# Autodesk Inventor assembly: Gear central part
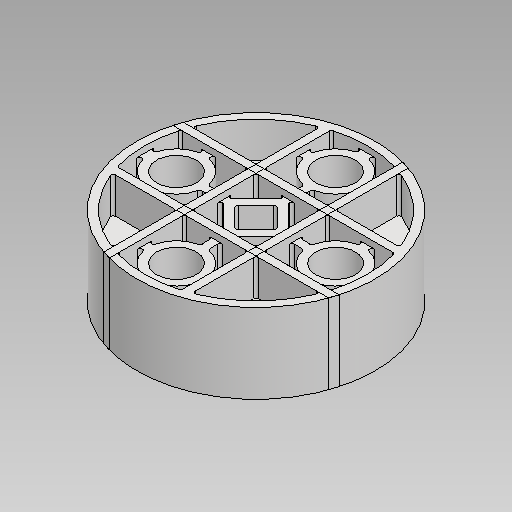
[picture p0: Inventor's stored thumbnail of the model, 512x512]
Saved by Autodesk Inventor 2020 (Build 240168000, 168)
## iProperties
Created: 2019-05-06
Part Number: Gear central part
Document SubType Name: Assembly
Designer: Varga Daniel
Author: Varga Daniel
## Documents named in this file (3)
- C:\!_Dani\!_cloud\OneDrive\!_munka\Revolution\StructuralParts\Gears\Gear central part.iam
- C:\!_Dani\!_cloud\OneDrive\!_munka\Revolution\StructuralParts\Gears\Gear side part.ipt
- C:\!_Dani\!_cloud\OneDrive\!_munka\Revolution\StructuralParts\Beams\Axle Beams\Axle beam base.ipt
## Components (5 placed, 2 different names)
1. Gear side part:1 — Flush:4, Flush:8, Flush:11
2. Gear side part:2 — Flush:2, Flush:6, Flush:9
3. Gear side part:3 — Flush:1, Flush:5, Flush:12
4. Gear side part:4 — Flush:3, Flush:7, Flush:10
5. Axle beam base:1 — Flush:1, Flush:2, Flush:3, Flush:4, Flush:5, Flush:6, Flush:7, Flush:8, Flush:9, Flush:10, Flush:11, Flush:12, Mate:1, Mate:2, Flush:13
## Relationships (15: Flush 13, Mate 2)
- Flush:1: Gear side part:3 ↔ Axle beam base:1
- Flush:2: Gear side part:2 ↔ Axle beam base:1
- Flush:3: Gear side part:4 ↔ Axle beam base:1
- Flush:4: Gear side part:1 ↔ Axle beam base:1
- Flush:5: Gear side part:3 ↔ Axle beam base:1
- Flush:6: Gear side part:2 ↔ Axle beam base:1
- Flush:7: Gear side part:4 ↔ Axle beam base:1
- Flush:8: Gear side part:1 ↔ Axle beam base:1
- Flush:9: Gear side part:2 ↔ Axle beam base:1
- Flush:10: Gear side part:4 ↔ Axle beam base:1
- Flush:11: Gear side part:1 ↔ Axle beam base:1
- Flush:12: Gear side part:3 ↔ Axle beam base:1
- Mate:1: Axle beam base:1
- Mate:2: Axle beam base:1
- Flush:13: Axle beam base:1
